# Autodesk Inventor assembly: Y_Axes
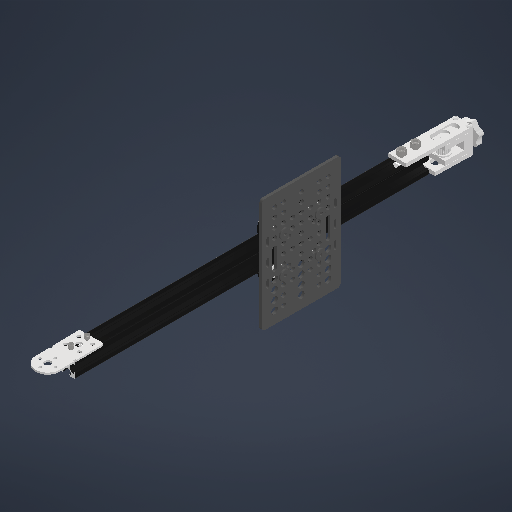
[picture p0: Inventor's stored thumbnail of the model, 512x512]
Saved by Autodesk Inventor 2027.1 (Build 311270010, 270A)
## iProperties
Created: 2026-10-02
Part Number: Y_Axes
Document SubType Name: Assembly
Designer: SDS Scholar
Author: SDS Scholar
## Documents named in this file (9)
- E:\Apps\AutodeskInventor\University\MCT333_Design1\Y_Axis.iam
- E:\Apps\AutodeskInventor\University\MCT333_Design1\OnTheShelf\AluminumExtrusion\AluminiumExtrusion2020\Y_axis.ipt
- E:\Apps\AutodeskInventor\University\MCT333_Design1\OnTheShelf\GT2BeltTensioner\2020 Belt Tensioner G_K\2020 Belt Tensioner G_K.ipt
- E:\Apps\AutodeskInventor\University\MCT333_Design1\OnTheShelf\slider-t-nut-for-2020-and-3030-aluminium-profile\2020\Slider T-Nut for 2020 - M5\Slider T-Nut for 2020 - M5.ipt
- C:\Users\SDS Scholar\Documents\Inventor\Content Center Files\R2027\en-US\SS-ISO 4762\ISO 4762 - M5 x 12SS-ISO.ipt
- E:\Apps\AutodeskInventor\University\MCT333_Design1\OnTheShelf\MotorMountPlate\motor holder bracket.ipt
- E:\Apps\AutodeskInventor\University\MCT333_Design1\OnTheShelf\slider-t-nut-for-2020-and-3030-aluminium-profile\2020\Slider T-Nut for 2020 - M3\Slider T-Nut for 2020 - M3.ipt
- C:\Users\SDS Scholar\Documents\Inventor\Content Center Files\R2027\en-US\ISO 4762(2)\ISO 4762 - M3 x 10ISO.ipt
- E:\Apps\AutodeskInventor\University\MCT333_Design1\OnTheShelf\VSoltGantrySetAllSizes\Inventor\40mm Gantry Set universal.iam
## Components (12 placed, 8 different names)
1. Y_axis:1 — Mate:1, Mate:2, Mate:3, Mate:4, Mate:5, Mate:6, Mate:7, Mate:10, Mate:13, Mate:14, Flush:1, Mate:15, Mate:16, Mate:17, Mate:18, Mate:21, Mate:22, Mate:25, Flush:2, Tangent:1, Tangent:2, Tangent:3, Tangent:4
2. 40mm Gantry Set universal:1 [sub-assembly] — Tangent:1, Tangent:2, Tangent:3, Tangent:4
3. 2020 Belt Tensioner G_K:1 — Mate:8, Mate:11, Mate:14
4. SS ISO 4762 M5 x 12:1 — Mate:11, Mate:12, Mate:13
5. SS ISO 4762 M5 x 12:2 — Mate:8, Mate:9, Mate:10
6. Slider T-Nut for 2020 - M5:1 — Mate:4, Mate:5, Mate:9, Flush:1
7. Slider T-Nut for 2020 - M5:2 — Mate:6, Mate:7, Mate:12
8. motor holder bracket:1 — Mate:19, Mate:22, Mate:23
9. Slider T-Nut for 2020 - M3:1 — Mate:15, Mate:16, Mate:20
10. Slider T-Nut for 2020 - M3:2 — Mate:17, Mate:18, Mate:24, Flush:2
11. ISO 4762 M3 x 10:1 — Mate:23, Mate:24, Mate:25
12. ISO 4762 M3 x 10:2 — Mate:19, Mate:20, Mate:21
## Relationships (31: Mate 25, Tangent 4, Flush 2)
- Mate:1: Y_axis:1
- Mate:2: Y_axis:1
- Mate:3: Y_axis:1
- Mate:4: Y_axis:1 ↔ Slider T-Nut for 2020 - M5:1
- Mate:5: Y_axis:1 ↔ Slider T-Nut for 2020 - M5:1
- Mate:6: Y_axis:1 ↔ Slider T-Nut for 2020 - M5:2
- Mate:7: Y_axis:1 ↔ Slider T-Nut for 2020 - M5:2
- Mate:8: 2020 Belt Tensioner G_K:1 ↔ SS ISO 4762 M5 x 12:2
- Mate:9: SS ISO 4762 M5 x 12:2 ↔ Slider T-Nut for 2020 - M5:1
- Mate:10: Y_axis:1 ↔ SS ISO 4762 M5 x 12:2
- Mate:11: 2020 Belt Tensioner G_K:1 ↔ SS ISO 4762 M5 x 12:1
- Mate:12: SS ISO 4762 M5 x 12:1 ↔ Slider T-Nut for 2020 - M5:2
- Mate:13: Y_axis:1 ↔ SS ISO 4762 M5 x 12:1
- Mate:14: Y_axis:1 ↔ 2020 Belt Tensioner G_K:1
- Flush:1: Y_axis:1 ↔ Slider T-Nut for 2020 - M5:1
- Mate:15: Y_axis:1 ↔ Slider T-Nut for 2020 - M3:1
- Mate:16: Y_axis:1 ↔ Slider T-Nut for 2020 - M3:1
- Mate:17: Y_axis:1 ↔ Slider T-Nut for 2020 - M3:2
- Mate:18: Y_axis:1 ↔ Slider T-Nut for 2020 - M3:2
- Mate:19: motor holder bracket:1 ↔ ISO 4762 M3 x 10:2
- Mate:20: Slider T-Nut for 2020 - M3:1 ↔ ISO 4762 M3 x 10:2
- Mate:21: Y_axis:1 ↔ ISO 4762 M3 x 10:2
- Mate:22: Y_axis:1 ↔ motor holder bracket:1
- Mate:23: motor holder bracket:1 ↔ ISO 4762 M3 x 10:1
- Mate:24: Slider T-Nut for 2020 - M3:2 ↔ ISO 4762 M3 x 10:1
- Mate:25: Y_axis:1 ↔ ISO 4762 M3 x 10:1
- Flush:2: Y_axis:1 ↔ Slider T-Nut for 2020 - M3:2
- Tangent:1: Y_axis:1 ↔ 40mm Gantry Set universal:1
- Tangent:2: Y_axis:1 ↔ 40mm Gantry Set universal:1
- Tangent:3: Y_axis:1 ↔ 40mm Gantry Set universal:1
- Tangent:4: Y_axis:1 ↔ 40mm Gantry Set universal:1
